# Autodesk Inventor assembly: Aug hit
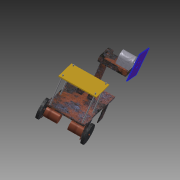
[picture p0: Inventor's stored thumbnail of the model, 180x180]
Saved by Autodesk Inventor 2014 (Build 180170000, 170)
## iProperties
Created: 2014-11-30
Part Number: Aug hit
Document SubType Name: Assembly
Designer: ph1140784
Author: ph1140784
## Documents named in this file (11)
- C:\Users\ph1140784\Documents\Aug hit final 2\Aug hit.iam
- C:\Users\ph1140784\Documents\Aug hit final 2\robot chasis.ipt
- C:\Users\ph1140784\Documents\Aug hit final 2\motor.ipt
- C:\Users\ph1140784\Documents\Aug hit final 2\screw.ipt
- C:\Users\ph1140784\Documents\Aug hit final 2\top panel.ipt
- C:\Users\ph1140784\Documents\Aug hit final 2\servo.ipt
- C:\Users\ph1140784\Documents\Aug hit final 2\marker plate.ipt
- C:\Users\ph1140784\Documents\Aug hit final 2\wheel 1.ipt
- C:\Users\ph1140784\Documents\Aug hit final 2\motor_MIR.ipt
- C:\Users\ph1140784\Documents\Aug hit final 2\wheel 1_MIR.ipt
- C:\Users\ph1140784\Documents\Aug hit final 2\chasis wheel.ipt
## Components (13 placed, 10 different names)
1. robot chasis:1 — Mate:7, Mate:8, Mate:9, Mate:10, Flush:1, Flush:2, Flush:3, Flush:4, Mate:35, Mate:36, Mate:38, Mate:39, Mate:48, Flush:16, Flush:17, Mate:49, Mate:50
2. motor:2 — Mate:23, Mate:35, Flush:14, Mate:36
3. screw:1 — Mate:9, Flush:3
4. screw:2 — Mate:8, Flush:1, Mate:32, Flush:13
5. screw:3 — Mate:10, Flush:4, Mate:33
6. screw:4 — Mate:7, Flush:2
7. servo:1 — Mate:45, Mate:46, Mate:48, Flush:16, Flush:17
8. marker plate:1 — Mate:45, Mate:46
9. wheel 1:2 — Mate:23, Flush:14
10. top panel:2 — Mate:32, Mate:33, Flush:13
11. motor_MIR:1 — Flush:15, Mate:37, Mate:38, Mate:39
12. wheel 1_MIR:1 — Flush:15, Mate:37
13. chasis wheel:1 — Mate:49, Mate:50
## Relationships (26: Mate 17, Flush 9)
- Mate:7: robot chasis:1 ↔ screw:4
- Mate:8: robot chasis:1 ↔ screw:2
- Mate:9: robot chasis:1 ↔ screw:1
- Mate:10: robot chasis:1 ↔ screw:3
- Flush:1: robot chasis:1 ↔ screw:2
- Flush:2: robot chasis:1 ↔ screw:4
- Flush:3: robot chasis:1 ↔ screw:1
- Flush:4: robot chasis:1 ↔ screw:3
- Mate:23: motor:2 ↔ wheel 1:2
- Mate:32: screw:2 ↔ top panel:2
- Mate:33: screw:3 ↔ top panel:2
- Flush:13 (5 mm): screw:2 ↔ top panel:2
- Mate:35: robot chasis:1 ↔ motor:2
- Flush:14 (2 mm): motor:2 ↔ wheel 1:2
- Mate:36: robot chasis:1 ↔ motor:2
- Flush:15 (2 mm): motor_MIR:1 ↔ wheel 1_MIR:1
- Mate:37: motor_MIR:1 ↔ wheel 1_MIR:1
- Mate:38: robot chasis:1 ↔ motor_MIR:1
- Mate:39: robot chasis:1 ↔ motor_MIR:1
- Mate:45: servo:1 ↔ marker plate:1
- Mate:46: servo:1 ↔ marker plate:1
- Mate:48: robot chasis:1 ↔ servo:1
- Flush:16: robot chasis:1 ↔ servo:1
- Flush:17 (9 mm): robot chasis:1 ↔ servo:1
- Mate:49: robot chasis:1 ↔ chasis wheel:1
- Mate:50: robot chasis:1 ↔ chasis wheel:1
